# Autodesk Inventor assembly: back_brace
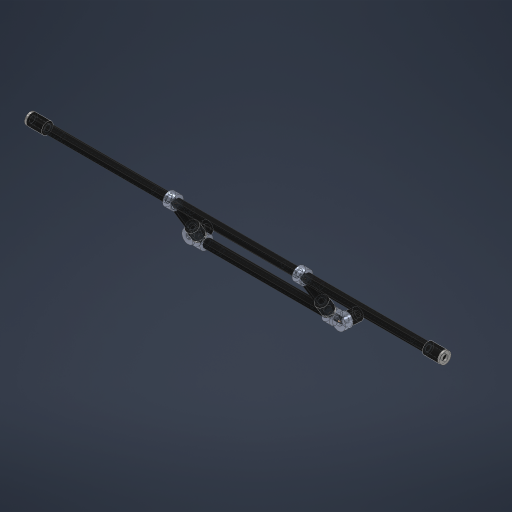
[picture p0: Inventor's stored thumbnail of the model, 512x512]
Saved by Autodesk Inventor 2024 (Build 280153000, 153)
## iProperties
Created: 2023-09-17
Part Number: back_brace
Document SubType Name: Assembly
Designer: Averey Ku
Author: Averey Ku
## Documents named in this file (12)
- D:\vex_robotics\hardware\cad\scrap_v0.1\chassis\back_brace.iam
- D:\vex_robotics\hardware\cad\VEX-CAD-Inventor-1.41\Structure\Standoff\Standoff 4.00.ipt
- D:\vex_robotics\hardware\cad\VEX-CAD-Inventor-1.41\Structure\Standoff.ipt
- D:\vex_robotics\hardware\cad\VEX-CAD-Inventor-1.41\Motion\Shaft LS\Shaft Collar ipts\Shaft Collar No Screw.ipt
- D:\vex_robotics\hardware\cad\VEX-CAD-Inventor-1.41\Motion\Spacers\Spacer Nylon .375 OD\NSpacer .375 OD x .375.ipt
- D:\vex_robotics\hardware\cad\VEX-CAD-Inventor-1.41\Motion\Spacers\Spacer Nylon .375 OD.ipt
- D:\vex_robotics\hardware\cad\VEX-CAD-Inventor-1.41\Structure\Standoff\Standoff 1.00.ipt
- D:\vex_robotics\hardware\cad\VEX-CAD-Inventor-1.41\Motion\Spacers\Washer Teflon\TWasher .375 OD x .04000.ipt
- D:\vex_robotics\hardware\cad\VEX-CAD-Inventor-1.41\Motion\Spacers\Washer Teflon.ipt
- D:\vex_robotics\hardware\cad\VEX-CAD-Inventor-1.41\Motion\Spacers\Washer Steel\SWasher .375 OD x .062500.ipt
- D:\vex_robotics\hardware\cad\VEX-CAD-Inventor-1.41\Motion\Spacers\Washer Steel.ipt
- D:\vex_robotics\hardware\cad\VEX-CAD-Inventor-1.41\Motion\Spacers\Spacer Nylon .375 OD\NSpacer .375 OD x .500.ipt
## Components (24 placed, 7 different names)
1. Standoff 4.00:1 — Insert:1, Insert:2
2. Shaft Collar No Screw:1 — Insert:1, Insert:4, Insert:14
3. Shaft Collar No Screw:2 — Insert:2, Insert:3, Insert:10
4. Shaft Collar No Screw:3 — Insert:3, Insert:5
5. Shaft Collar No Screw:4 — Insert:4, Insert:6
6. NSpacer .375 OD x .375:1 — Insert:5, Angle:1
7. NSpacer .375 OD x .375:2 — Insert:6, Angle:1
8. Standoff 1.00:2 — Insert:16
9. NSpacer .375 OD x .375:3
10. TWasher .375 OD x .04000:1
11. TWasher .375 OD x .04000:2 — Insert:10
12. Standoff 1.00:3 — Insert:15
13. NSpacer .375 OD x .375:4
14. TWasher .375 OD x .04000:3
15. TWasher .375 OD x .04000:4 — Insert:14
16. Shaft Collar No Screw:5 — Insert:15, Insert:17, Insert:20
17. Shaft Collar No Screw:6 — Insert:16, Insert:18, Insert:19
18. Standoff 4.00:4 — Insert:17, Insert:18
19. Standoff 4.00:5 — Insert:19, Insert:23
20. Standoff 4.00:6 — Insert:20, Insert:24
21. SWasher .375 OD x .062500:1
22. NSpacer .375 OD x .500:5 — Insert:24
23. SWasher .375 OD x .062500:2
24. NSpacer .375 OD x .500:6 — Insert:23
## Relationships (25: Insert 24, Angle 1)
- Insert:1: Standoff 4.00:1 ↔ Shaft Collar No Screw:1
- Insert:2: Standoff 4.00:1 ↔ Shaft Collar No Screw:2
- Insert:3: Shaft Collar No Screw:2 ↔ Shaft Collar No Screw:3
- Insert:4: Shaft Collar No Screw:1 ↔ Shaft Collar No Screw:4
- Insert:5: Shaft Collar No Screw:3 ↔ NSpacer .375 OD x .375:1
- Insert:6: Shaft Collar No Screw:4 ↔ NSpacer .375 OD x .375:2
- [Insert]: TWasher .375 OD x .04000:1 ↔ TWasher .375 OD x .04000:2
- [Insert]: NSpacer .375 OD x .375:3 ↔ TWasher .375 OD x .04000:1
- [Insert]: Standoff 1.00:2 ↔ NSpacer .375 OD x .375:3
- Insert:10: Shaft Collar No Screw:2 ↔ TWasher .375 OD x .04000:2
- [Insert]: TWasher .375 OD x .04000:3 ↔ TWasher .375 OD x .04000:4
- [Insert]: NSpacer .375 OD x .375:4 ↔ TWasher .375 OD x .04000:3
- [Insert]: Standoff 1.00:3 ↔ NSpacer .375 OD x .375:4
- Insert:14: Shaft Collar No Screw:1 ↔ TWasher .375 OD x .04000:4
- Insert:15: Standoff 1.00:3 ↔ Shaft Collar No Screw:5
- Insert:16: Standoff 1.00:2 ↔ Shaft Collar No Screw:6
- Insert:17: Shaft Collar No Screw:5 ↔ Standoff 4.00:4
- Insert:18: Shaft Collar No Screw:6 ↔ Standoff 4.00:4
- Insert:19: Shaft Collar No Screw:6 ↔ Standoff 4.00:5
- Insert:20: Shaft Collar No Screw:5 ↔ Standoff 4.00:6
- [Insert]: SWasher .375 OD x .062500:1 ↔ NSpacer .375 OD x .500:5
- [Insert]: SWasher .375 OD x .062500:2 ↔ NSpacer .375 OD x .500:6
- Insert:23: Standoff 4.00:5 ↔ NSpacer .375 OD x .500:6
- Insert:24: Standoff 4.00:6 ↔ NSpacer .375 OD x .500:5
- Angle:1 (0 deg): NSpacer .375 OD x .375:1 ↔ NSpacer .375 OD x .375:2
## Named parameters: d10_d12 = 0 mm, d11_d13 = 0 mm, d15_d14 = 0 mm, d24_d29 = 0 mm
